# Autodesk Inventor assembly: Montagem6
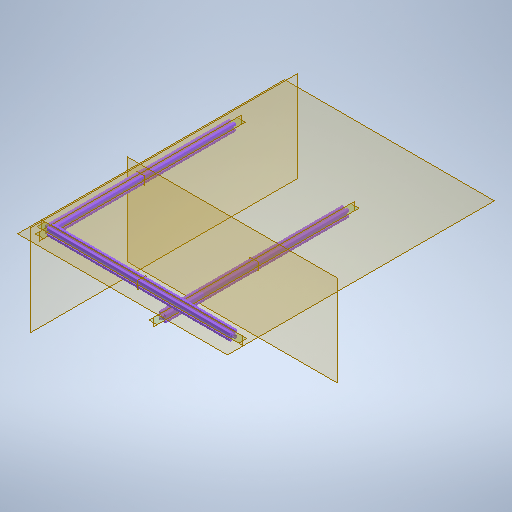
[picture p0: Inventor's stored thumbnail of the model, 512x512]
Saved by Autodesk Inventor 2025.2 (Build 292293000, 293)
## iProperties
Created: 2025-03-28
Part Number: Montagem6
Document SubType Name: Assembly
Designer: Formação
Author: Formação
## Documents named in this file (2)
- C:\Users\Formação\Documents\Inventor\Sessão_25_03_25\Montagem6.iam
- C:\Users\Formação\Documents\Inventor\Sessão_25_03_25\Peça2.ipt
## Components (3 placed, 1 different names)
1. Peça2:1 — Alinhado:1, Coincidente:1, Coincidente:2, Coincidente:3, Coincidente:4
2. Peça2:2
3. Peça2:3 — Coincidente:3, Coincidente:4
## Relationships (5: Mate 4, Flush 1)
- Alinhado:1 [Flush]: Peça2:1
- Coincidente:1 [Mate]: Peça2:1
- Coincidente:2 [Mate]: Peça2:1
- Coincidente:3 [Mate]: Peça2:1 ↔ Peça2:3
- Coincidente:4 [Mate]: Peça2:1 ↔ Peça2:3
